# Autodesk Inventor assembly: tandwiel
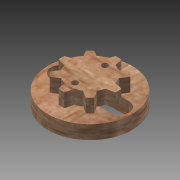
[picture p0: Inventor's stored thumbnail of the model, 180x180]
Saved by Autodesk Inventor 2015 (Build 190159000, 159)
## iProperties
Created: 2016-01-31
Part Number: tandwiel
Document SubType Name: Assembly
Designer: david
Author: david
## Documents named in this file (3)
- Z:\gip\Inventor\generatie 7\motor\tandwiel\tandwiel.iam
- Z:\gip\Inventor\generatie 7\motor\tandwiel\1.ipt
- Z:\gip\Inventor\generatie 7\motor\tandwiel\tandwiel(ja).ipt
## Components (4 placed, 2 different names)
1. 1:1 — Mate:1, Mate:2, Flush:1
2. 1:2 — Mate:1, Mate:2, Flush:1, Flush:2, Flush:3, Flush:4
3. tandwiel(ja):1 — Flush:2, Flush:3, Flush:4, Mate:3, Mate:4, Flush:5
4. tandwiel(ja):2 — Mate:3, Mate:4, Flush:5
## Relationships (9: Flush 5, Mate 4)
- Mate:1: 1:1 ↔ 1:2
- Mate:2: 1:1 ↔ 1:2
- Flush:1: 1:1 ↔ 1:2
- Flush:2: 1:2 ↔ tandwiel(ja):1
- Flush:3: 1:2 ↔ tandwiel(ja):1
- Flush:4: 1:2 ↔ tandwiel(ja):1
- Mate:3: tandwiel(ja):1 ↔ tandwiel(ja):2
- Mate:4: tandwiel(ja):1 ↔ tandwiel(ja):2
- Flush:5: tandwiel(ja):1 ↔ tandwiel(ja):2
